# Autodesk Inventor assembly: seperatorSheet
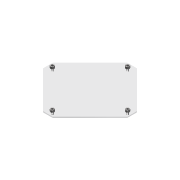
[picture p0: Inventor's stored thumbnail of the model, 180x180]
Saved by Autodesk Inventor 2017 (Build 210142000, 142)
## iProperties
Created: 2017-01-08
Part Number: seperatorSheet
Document SubType Name: Assembly
Designer: sawaiz
Author: sawaiz
## Documents named in this file (3)
- C:\Users\sawaiz\oneDrive\projects\muonTelescope\frame\separator\seperatorSheet.iam
- C:\Users\sawaiz\oneDrive\projects\muonTelescope\frame\separator\separatingPanels.ipt
- C:\Users\sawaiz\oneDrive\projects\muonTelescope\frame\brackets\m5x6.ipt
## Components (5 placed, 2 different names)
1. separatingPanels:1 — Mate:1, Mate:2, Mate:3, Mate:4, Mate:5
2. m5x6:1 — Mate:1, Flush:1, Flush:2
3. m5x6:2 — Mate:2, Flush:2, Flush:3
4. m5x6:3 — Mate:3, Flush:3, Mate:5
5. m5x6:4 — Mate:4, Flush:1
## Relationships (8: Mate 5, Flush 3)
- Mate:1: separatingPanels:1 ↔ m5x6:1
- Mate:2: separatingPanels:1 ↔ m5x6:2
- Mate:3: separatingPanels:1 ↔ m5x6:3
- Mate:4: separatingPanels:1 ↔ m5x6:4
- Flush:1: m5x6:1 ↔ m5x6:4
- Flush:2: m5x6:1 ↔ m5x6:2
- Flush:3: m5x6:2 ↔ m5x6:3
- Mate:5: separatingPanels:1 ↔ m5x6:3
